# Autodesk Inventor assembly: arm two
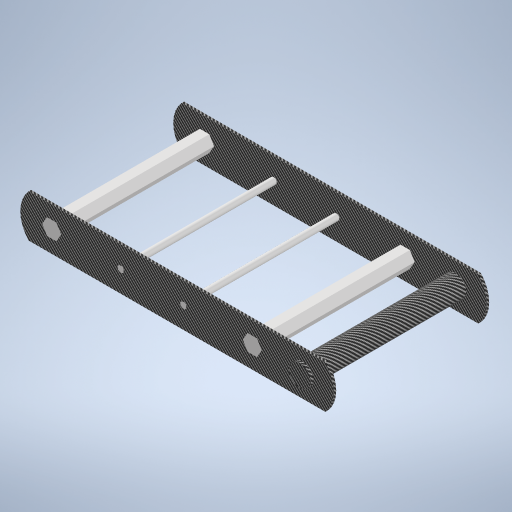
[picture p0: Inventor's stored thumbnail of the model, 512x512]
Saved by Autodesk Inventor 2023 (Build 270158000, 158)
## iProperties
Created: 2023-01-03
Part Number: arm two
Document SubType Name: Assembly
Designer: victo
Author: victo
## Documents named in this file (5)
- C:\Users\victo\OneDrive\Documents\rcr\completely new\arm two.iam
- C:\Users\victo\OneDrive\Documents\rcr\completely new\new arm plate.ipt
- C:\Users\victo\OneDrive\Documents\rcr\completely new\hex shaft.ipt
- C:\Users\victo\OneDrive\Documents\rcr\completely new\new rotary shaft.ipt
- C:\Users\victo\OneDrive\Documents\rcr\completely new\big rotary shaft.ipt
## Components (7 placed, 4 different names)
1. new arm plate:1 — Rotational:3, Rotational:4
2. new arm plate:2
3. hex shaft:1
4. hex shaft:2
5. new rotary shaft:1
6. new rotary shaft:2
7. big rotary shaft:1 — Rotational:3, Rotational:4
## Relationships (7: RevoluteJoint 4, WeldJoint 3)
- [WeldJoint]: new arm plate:1 ↔ hex shaft:1
- [WeldJoint]: new arm plate:2 ↔ hex shaft:1
- [WeldJoint]: new arm plate:1 ↔ hex shaft:2
- [RevoluteJoint]: new arm plate:1 ↔ new rotary shaft:1
- [RevoluteJoint]: new arm plate:1 ↔ new rotary shaft:2
- Rotational:3 [RevoluteJoint]: new arm plate:1 ↔ big rotary shaft:1
- Rotational:4 [RevoluteJoint] (-3.048 mm): new arm plate:1 ↔ big rotary shaft:1
## Named parameters: d0_d6 = 0 mm
